# Autodesk Inventor assembly: Kepler_Vibe_XL
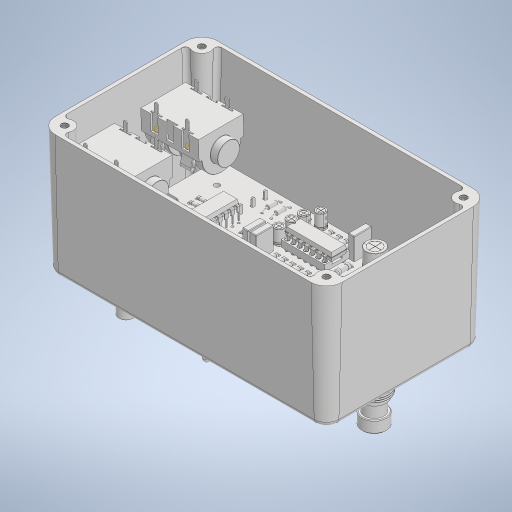
[picture p0: Inventor's stored thumbnail of the model, 512x512]
Saved by Autodesk Inventor 2023 (Build 270158030, 158C)
## iProperties
Created: 2022-11-10
Part Number: Kepler_Vibe_XL
Document SubType Name: Assembly
Designer: Imogen Heard
Author: Imogen Heard
## iProperties of the stored document 6_3 Jack contact_01.ipt
Created: 2015-03-06
Part Number: 6_3 Jack contact_01
Material: Generic
Document SubType Name: Modeling
Designer: Imogen Heard
Density: 1 g/cm^3
Appearance: Default
Author: Imogen Heard
Revision Number: ANY
## iProperties of the stored document DJ Jack 2,1mm panel mount v1.ipt
Created: 2022-11-14
Part Number: DJ Jack 2,1mm panel mount v1
Material: Generic
Document SubType Name: Modeling
Designer: Imogen Heard
Density: 1 g/cm^3
Appearance: Default
Author: Imogen Heard
## iProperties of the stored document 6.35mm Mono Jack Socket Connector.iam
Created: 2015-03-06
Part Number: 6.35mm Mono Jack Socket Connector
Description: STEP AP203
Document SubType Name: Assembly
Designer: Imogen Heard
Sending System: SolidWorks 2014
Preprocessor: SwSTEP 2.0
Title: 6.35mm Mono Jack Socket Connector.STEP
Author: NoiroSM250
Revision Number: ANY
## iProperties of the stored document dc 022B  jack 2.1mm.iam
Created: 2017-05-30
Part Number: dc jack 2.1mm v5
Document SubType Name: Assembly
Designer: Imogen Heard
Sending System: Autodesk Translation Framework v6.1.1.50
Preprocessor: ST-DEVELOPER v16.13
Title: /Users/paulo/Desktop/dc 022B  jack 2.1mm.step
## iProperties of the stored document 6_3 Jack contact_02.ipt
Created: 2015-03-06
Part Number: 6_3 Jack contact_02
Material: Generic
Document SubType Name: Modeling
Designer: Imogen Heard
Density: 1 g/cm^3
Appearance: Default
Author: Imogen Heard
Revision Number: ANY
## iProperties of the stored document 6_3 Jack body.ipt
Created: 2015-03-06
Part Number: 6_3 Jack body
Material: Generic
Document SubType Name: Modeling
Designer: Imogen Heard
Density: 1 g/cm^3
Appearance: Default
Author: Imogen Heard
Revision Number: ANY
## iProperties of the stored document Nut.ipt
Created: 2015-03-06
Part Number: Nut
Material: Generic
Document SubType Name: Modeling
Designer: Imogen Heard
Density: 1 g/cm^3
Appearance: Default
Author: Imogen Heard
Revision Number: ANY
## Documents named in this file (12)
- C:\Users\dheard\Documents\Inventor\Inventor_Projects\Electronics Projects\Kepler_Vibe_XL.iam
- C:\Users\dheard\Documents\Inventor\Inventor_Projects\Enclosures\Die Cast Box.ipt
- C:\Users\dheard\Documents\Inventor\Inventor_Projects\Electronics Projects\Kepler_Vibe_PCB_v2.ipt
- **C:\Users\dheard\Documents\Inventor\Inventor_Projects\Electronics Projects\Kepler_Vibe_XL.iam*LocalDocs*xAaaaazcaAaaaaaaaAaaaqzghLf*6.35mm Mono Jack Socket Connector.iam
- **C:\Users\dheard\Documents\Inventor\Inventor_Projects\Electronics Projects\Kepler_Vibe_XL.iam*LocalDocs*xAaaaatdaAaaaaaaaAaaaqpqwCe*dc 022B  jack 2.1mm.iam
- **C:\Users\dheard\Documents\Inventor\Inventor_Projects\Electronics Projects\Kepler_Vibe_XL.iam*LocalDocs*xAaaaapbaAaaaaaaaAaaaq23cSg*6_3 Jack contact_01.ipt
- **C:\Users\dheard\Documents\Inventor\Inventor_Projects\Electronics Projects\Kepler_Vibe_XL.iam*LocalDocs*xAaaaa4baAaaaaaaaAaaaaw1nWa*DJ Jack 2,1mm panel mount v1.ipt
- **C:\Users\dheard\Documents\Inventor\Inventor_Projects\Electronics Projects\Kepler_Vibe_XL.iam*LocalDocs*xAaaaq1baAaaaaaaaAaaaahcpEe*6_3 Jack body.ipt
- **C:\Users\dheard\Documents\Inventor\Inventor_Projects\Electronics Projects\Kepler_Vibe_XL.iam*LocalDocs*xAaaaqscaAaaaaaaaAaaaqe1lKg*Nut.ipt
- **C:\Users\dheard\Documents\Inventor\Inventor_Projects\Electronics Projects\Kepler_Vibe_XL.iam*LocalDocs*xAaaaqpcaAaaaaaaaAaaaqb54Hb*6_3 Jack contact_02.ipt
- C:\Users\dheard\Documents\0000.KiCad\6.0\3rdparty\000_Immo_3D_models\6-35mm-mono-jack-socket-connector-1.snapshot.7\6.35mm Mono Jack Socket Connector.STEP
- C:\Users\dheard\Documents\0000.KiCad\6.0\3rdparty\000_Immo_3D_models\dc-jack-0022b-2-1mm-panel-mount-1.snapshot.3\dc 022B  jack 2.1mm.step
## Components (5 placed, 4 different names)
1. Die Cast Box:1 — Mate:1, Mate:2, Mate:3, Mate:4, Mate:5, Mate:6
2. Kepler_Vibe_PCB_v2:1 — Mate:1, Mate:2, Mate:3
3. 6.35mm Mono Jack Socket Connector:2 [sub-assembly] — Flush:1, Flush:2
4. 6.35mm Mono Jack Socket Connector:3 [sub-assembly] — Flush:1, Mate:4, Mate:6, Flush:2
5. dc 022B  jack 2.1mm:1 [sub-assembly] — Mate:5
## Relationships (8: Mate 6, Flush 2)
- Mate:1: Die Cast Box:1 ↔ Kepler_Vibe_PCB_v2:1
- Mate:2 (2 mm): Die Cast Box:1 ↔ Kepler_Vibe_PCB_v2:1
- Mate:3 (37 mm): Die Cast Box:1 ↔ Kepler_Vibe_PCB_v2:1
- Flush:1: 6.35mm Mono Jack Socket Connector:2 ↔ 6.35mm Mono Jack Socket Connector:3
- Mate:4: Die Cast Box:1 ↔ 6.35mm Mono Jack Socket Connector:3
- Mate:5: Die Cast Box:1 ↔ dc 022B  jack 2.1mm:1
- Mate:6 (10 mm): Die Cast Box:1 ↔ 6.35mm Mono Jack Socket Connector:3
- Flush:2: 6.35mm Mono Jack Socket Connector:2 ↔ 6.35mm Mono Jack Socket Connector:3
